# Autodesk Inventor assembly: Schwingforderer SF-TAG-N 250-20-105 R Al with loose ground(SRL-N250 AL)
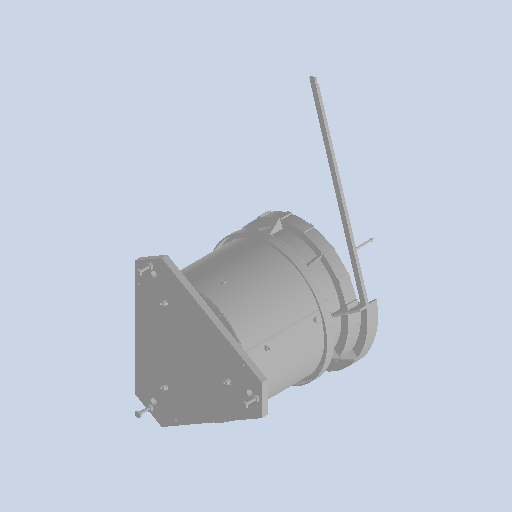
[picture p0: Inventor's stored thumbnail of the model, 512x512]
Saved by Autodesk Inventor 2025.2 (Build 292293000, 293)
## iProperties
Category: PARTsolutions
Company: RNA
Created: 2025-06-16
Part Number: Schwingforderer SF-TAG-N 250-20-105 R Al with loose ground(SRL-N250 AL)
Catalog Web Link: www.cadenas.de
Description: 250-Vibratory Bowl Feeder
Vendor: RNA
Document SubType Name: Assembly
Designer: psAdmin
Manufacturer: RNA
Mass: 8037.77 g
Surface Area: 14728.5 cm^2
Volume: 8037.77 cm^3
Density: 1 g/cm^3
PSOL_IDENT_0: {$CADENAS_DATA/23d-libs/rna/schwingfoerderer/bg_250.prj},262 {STYP=ASS},{VTYP=3D},{NB=Schwingfordere
PSOL_IDENT_1: r SF-TAG-N 250-20-105 R Al with loose ground(SRL-N250 AL)},{LINA=SF-TAG-N 250-20-105 R Al with loose
PSOL_IDENT_2: ground},{NN=250},{DATE=06.06.2017 07:12:53},{GEOMDATE=02.06.2017 06:00:57},{VERSION=},{LINEID=120},
PSOL_IDENT_3: {WBVAR=},{WBNUMERIC=}  {NB=Schwingforderer SF-TAG-N 250-20-105 R Al with loose ground(SRL-N250 AL)},
PSOL_IDENT_4: {LINA=SF-TAG-N 250-20-105 R Al with loose ground},{KT=DUMMY},{NAME=SF-TAG-N 250-20-105 R Al with loo
PSOL_IDENT_5: se ground},{INAME=SF2dTAG2dN202502d202d10520R20Al20with20loose20ground},{SHA256=rV/3CrsxDAyYqkcBF+Y8
PSOL_IDENT_6: nExrJVCtF3b6/2GE7EfEZ3w=},{CNSORDERNO=SF-TAG-N 250-20-105 R Al with loose ground},{HIDE=0},{A=Stufen
PSOL_IDENT_7: },{B=250},{C=Radial oben},{D=ALU},{E=Lose eingelegt},{F=20},{G=TAG-N250-20-105},{H=ohne},{I=SRL-N250
PSOL_IDENT_8: AL},{J=SRC-N250},{K=USJ250}
NB: Schwingforderer SF-TAG-N 250-20-105 R Al with loose ground(SRL-N250 AL)
NN: 250
NT: Vibratory Bowl Feeder
NBSYN: Schwingforderer $CNSORDERNO.($I.)
LINA: SF-TAG-N 250-20-105 R Al with loose ground
CATALOG: Rhein-Nadel-Automation
CNSORDERNO: SF-TAG-N 250-20-105 R Al with loose ground
A: Stufen
B: 250
C: Radial oben
D: ALU
E: Lose eingelegt
F: 20
G: TAG-N250-20-105
H: ohne
I: SRL-N250 AL
J: SRC-N250
K: USJ250
SUPPLIER: RNA
ARTICLENO: Schwingforderer SF-TAG-N 250-20-105 R Al with loose ground(SRL-N250 AL)
BOMINFO: SF-TAG-N 250-20-105 R Al with loose ground
CREATOR: CADENAS GmbH
Title: SF-TAG-N 250-20-105 R Al with loose ground
Author: Cadenas PARTsolutions
Comments: Vibratory Bowl Feeder
## Documents named in this file (40)
- D:\Useless_Box\CAD-Paspa\Useless Box\Kaufteile\SF-TAG-N 250-20-105 R Al\Schwingforderer SF-TAG-N 250-20-105 R Al with loose ground(SRL-N250 AL).iam
- D:\Useless_Box\CAD-Paspa\Useless Box\Kaufteile\SF-TAG-N 250-20-105 R Al\Schwingforderer SF-TAG-N 250-20-105 R Al with loose ground(SRL-N250 AL)_PART1.ipt
- D:\Useless_Box\CAD-Paspa\Useless Box\Kaufteile\SF-TAG-N 250-20-105 R Al\Schwingforderer SF-TAG-N 250-20-105 R Al with loose ground(SRL-N250 AL)_PART2.ipt
- D:\Useless_Box\CAD-Paspa\Useless Box\Kaufteile\SF-TAG-N 250-20-105 R Al\Schwingforderer SF-TAG-N 250-20-105 R Al with loose ground(SRL-N250 AL)_PART3.ipt
- D:\Useless_Box\CAD-Paspa\Useless Box\Kaufteile\SF-TAG-N 250-20-105 R Al\Schwingforderer SF-TAG-N 250-20-105 R Al with loose ground(SRL-N250 AL)_PART4.ipt
- D:\Useless_Box\CAD-Paspa\Useless Box\Kaufteile\SF-TAG-N 250-20-105 R Al\Schwingforderer SF-TAG-N 250-20-105 R Al with loose ground(SRL-N250 AL)_PART5.ipt
- D:\Useless_Box\CAD-Paspa\Useless Box\Kaufteile\SF-TAG-N 250-20-105 R Al\Schwingforderer SF-TAG-N 250-20-105 R Al with loose ground(SRL-N250 AL)_PART6.ipt
- D:\Useless_Box\CAD-Paspa\Useless Box\Kaufteile\SF-TAG-N 250-20-105 R Al\Schwingforderer SF-TAG-N 250-20-105 R Al with loose ground(SRL-N250 AL)_PART7.ipt
- D:\Useless_Box\CAD-Paspa\Useless Box\Kaufteile\SF-TAG-N 250-20-105 R Al\Schwingforderer SF-TAG-N 250-20-105 R Al with loose ground(SRL-N250 AL)_PART8.ipt
- D:\Useless_Box\CAD-Paspa\Useless Box\Kaufteile\SF-TAG-N 250-20-105 R Al\Schwingforderer SF-TAG-N 250-20-105 R Al with loose ground(SRL-N250 AL)_PART9.ipt
- D:\Useless_Box\CAD-Paspa\Useless Box\Kaufteile\SF-TAG-N 250-20-105 R Al\Schwingforderer SF-TAG-N 250-20-105 R Al with loose ground(SRL-N250 AL)_PART10.ipt
- D:\Useless_Box\CAD-Paspa\Useless Box\Kaufteile\SF-TAG-N 250-20-105 R Al\Schwingforderer SF-TAG-N 250-20-105 R Al with loose ground(SRL-N250 AL)_PART11.ipt
- D:\Useless_Box\CAD-Paspa\Useless Box\Kaufteile\SF-TAG-N 250-20-105 R Al\Schwingforderer SF-TAG-N 250-20-105 R Al with loose ground(SRL-N250 AL)_PART12.ipt
- D:\Useless_Box\CAD-Paspa\Useless Box\Kaufteile\SF-TAG-N 250-20-105 R Al\Schwingforderer SF-TAG-N 250-20-105 R Al with loose ground(SRL-N250 AL)_PART13.ipt
- D:\Useless_Box\CAD-Paspa\Useless Box\Kaufteile\SF-TAG-N 250-20-105 R Al\Schwingforderer SF-TAG-N 250-20-105 R Al with loose ground(SRL-N250 AL)_PART14.ipt
- D:\Useless_Box\CAD-Paspa\Useless Box\Kaufteile\SF-TAG-N 250-20-105 R Al\Schwingforderer SF-TAG-N 250-20-105 R Al with loose ground(SRL-N250 AL)_PART15.ipt
- D:\Useless_Box\CAD-Paspa\Useless Box\Kaufteile\SF-TAG-N 250-20-105 R Al\Schwingforderer SF-TAG-N 250-20-105 R Al with loose ground(SRL-N250 AL)_PART16.ipt
- D:\Useless_Box\CAD-Paspa\Useless Box\Kaufteile\SF-TAG-N 250-20-105 R Al\Schwingforderer SF-TAG-N 250-20-105 R Al with loose ground(SRL-N250 AL)_PART17.ipt
- D:\Useless_Box\CAD-Paspa\Useless Box\Kaufteile\SF-TAG-N 250-20-105 R Al\Schwingforderer SF-TAG-N 250-20-105 R Al with loose ground(SRL-N250 AL)_PART18.ipt
- D:\Useless_Box\CAD-Paspa\Useless Box\Kaufteile\SF-TAG-N 250-20-105 R Al\Schwingforderer SF-TAG-N 250-20-105 R Al with loose ground(SRL-N250 AL)_PART19.ipt
- D:\Useless_Box\CAD-Paspa\Useless Box\Kaufteile\SF-TAG-N 250-20-105 R Al\Schwingforderer SF-TAG-N 250-20-105 R Al with loose ground(SRL-N250 AL)_PART20.ipt
- D:\Useless_Box\CAD-Paspa\Useless Box\Kaufteile\SF-TAG-N 250-20-105 R Al\Schwingforderer SF-TAG-N 250-20-105 R Al with loose ground(SRL-N250 AL)_PART21.ipt
- D:\Useless_Box\CAD-Paspa\Useless Box\Kaufteile\SF-TAG-N 250-20-105 R Al\Schwingforderer SF-TAG-N 250-20-105 R Al with loose ground(SRL-N250 AL)_PART22.ipt
- D:\Useless_Box\CAD-Paspa\Useless Box\Kaufteile\SF-TAG-N 250-20-105 R Al\Schwingforderer SF-TAG-N 250-20-105 R Al with loose ground(SRL-N250 AL)_PART23.ipt
- D:\Useless_Box\CAD-Paspa\Useless Box\Kaufteile\SF-TAG-N 250-20-105 R Al\Schwingforderer SF-TAG-N 250-20-105 R Al with loose ground(SRL-N250 AL)_PART24.ipt
- D:\Useless_Box\CAD-Paspa\Useless Box\Kaufteile\SF-TAG-N 250-20-105 R Al\Schwingforderer SF-TAG-N 250-20-105 R Al with loose ground(SRL-N250 AL)_PART25.ipt
- D:\Useless_Box\CAD-Paspa\Useless Box\Kaufteile\SF-TAG-N 250-20-105 R Al\Schwingforderer SF-TAG-N 250-20-105 R Al with loose ground(SRL-N250 AL)_PART26.ipt
- D:\Useless_Box\CAD-Paspa\Useless Box\Kaufteile\SF-TAG-N 250-20-105 R Al\Schwingforderer SF-TAG-N 250-20-105 R Al with loose ground(SRL-N250 AL)_PART27.ipt
- D:\Useless_Box\CAD-Paspa\Useless Box\Kaufteile\SF-TAG-N 250-20-105 R Al\Schwingforderer SF-TAG-N 250-20-105 R Al with loose ground(SRL-N250 AL)_PART28.ipt
- D:\Useless_Box\CAD-Paspa\Useless Box\Kaufteile\SF-TAG-N 250-20-105 R Al\Schwingforderer SF-TAG-N 250-20-105 R Al with loose ground(SRL-N250 AL)_PART29.ipt
- D:\Useless_Box\CAD-Paspa\Useless Box\Kaufteile\SF-TAG-N 250-20-105 R Al\Schwingforderer SF-TAG-N 250-20-105 R Al with loose ground(SRL-N250 AL)_PART30.ipt
- D:\Useless_Box\CAD-Paspa\Useless Box\Kaufteile\SF-TAG-N 250-20-105 R Al\Schwingforderer SF-TAG-N 250-20-105 R Al with loose ground(SRL-N250 AL)_PART31.ipt
- D:\Useless_Box\CAD-Paspa\Useless Box\Kaufteile\SF-TAG-N 250-20-105 R Al\Schwingforderer SF-TAG-N 250-20-105 R Al with loose ground(SRL-N250 AL)_PART32.ipt
- D:\Useless_Box\CAD-Paspa\Useless Box\Kaufteile\SF-TAG-N 250-20-105 R Al\Schwingforderer SF-TAG-N 250-20-105 R Al with loose ground(SRL-N250 AL)_PART33.ipt
- D:\Useless_Box\CAD-Paspa\Useless Box\Kaufteile\SF-TAG-N 250-20-105 R Al\Schwingforderer SF-TAG-N 250-20-105 R Al with loose ground(SRL-N250 AL)_PART34.ipt
- D:\Useless_Box\CAD-Paspa\Useless Box\Kaufteile\SF-TAG-N 250-20-105 R Al\Schwingforderer SF-TAG-N 250-20-105 R Al with loose ground(SRL-N250 AL)_PART35.ipt
- D:\Useless_Box\CAD-Paspa\Useless Box\Kaufteile\SF-TAG-N 250-20-105 R Al\Schwingforderer SF-TAG-N 250-20-105 R Al with loose ground(SRL-N250 AL)_PART36.ipt
- D:\Useless_Box\CAD-Paspa\Useless Box\Kaufteile\SF-TAG-N 250-20-105 R Al\Schwingforderer SF-TAG-N 250-20-105 R Al with loose ground(SRL-N250 AL)_PART37.ipt
- D:\Useless_Box\CAD-Paspa\Useless Box\Kaufteile\SF-TAG-N 250-20-105 R Al\Schwingforderer SF-TAG-N 250-20-105 R Al with loose ground(SRL-N250 AL)_PART38.ipt
- D:\Useless_Box\CAD-Paspa\Useless Box\Kaufteile\IB06A229_ind_sensor\IB06A229.ipt
## Components (39 placed, 39 different names)
1. Schwingforderer SF-TAG-N 250-20-105 R Al with loose ground(SRL-N250 AL)_PART1:1
2. Schwingforderer SF-TAG-N 250-20-105 R Al with loose ground(SRL-N250 AL)_PART2:1
3. Schwingforderer SF-TAG-N 250-20-105 R Al with loose ground(SRL-N250 AL)_PART3:1
4. Schwingforderer SF-TAG-N 250-20-105 R Al with loose ground(SRL-N250 AL)_PART4:1
5. Schwingforderer SF-TAG-N 250-20-105 R Al with loose ground(SRL-N250 AL)_PART5:1
6. Schwingforderer SF-TAG-N 250-20-105 R Al with loose ground(SRL-N250 AL)_PART6:1
7. Schwingforderer SF-TAG-N 250-20-105 R Al with loose ground(SRL-N250 AL)_PART7:1
8. Schwingforderer SF-TAG-N 250-20-105 R Al with loose ground(SRL-N250 AL)_PART8:1
9. Schwingforderer SF-TAG-N 250-20-105 R Al with loose ground(SRL-N250 AL)_PART9:1
10. Schwingforderer SF-TAG-N 250-20-105 R Al with loose ground(SRL-N250 AL)_PART10:1
11. Schwingforderer SF-TAG-N 250-20-105 R Al with loose ground(SRL-N250 AL)_PART11:1
12. Schwingforderer SF-TAG-N 250-20-105 R Al with loose ground(SRL-N250 AL)_PART12:1 — Passend:1
13. Schwingforderer SF-TAG-N 250-20-105 R Al with loose ground(SRL-N250 AL)_PART13:1
14. Schwingforderer SF-TAG-N 250-20-105 R Al with loose ground(SRL-N250 AL)_PART14:1
15. Schwingforderer SF-TAG-N 250-20-105 R Al with loose ground(SRL-N250 AL)_PART15:1
16. Schwingforderer SF-TAG-N 250-20-105 R Al with loose ground(SRL-N250 AL)_PART16:1
17. Schwingforderer SF-TAG-N 250-20-105 R Al with loose ground(SRL-N250 AL)_PART17:1
18. Schwingforderer SF-TAG-N 250-20-105 R Al with loose ground(SRL-N250 AL)_PART18:1
19. Schwingforderer SF-TAG-N 250-20-105 R Al with loose ground(SRL-N250 AL)_PART19:1
20. Schwingforderer SF-TAG-N 250-20-105 R Al with loose ground(SRL-N250 AL)_PART20:1
21. Schwingforderer SF-TAG-N 250-20-105 R Al with loose ground(SRL-N250 AL)_PART21:1
22. Schwingforderer SF-TAG-N 250-20-105 R Al with loose ground(SRL-N250 AL)_PART22:1
23. Schwingforderer SF-TAG-N 250-20-105 R Al with loose ground(SRL-N250 AL)_PART23:1
24. Schwingforderer SF-TAG-N 250-20-105 R Al with loose ground(SRL-N250 AL)_PART24:1
25. Schwingforderer SF-TAG-N 250-20-105 R Al with loose ground(SRL-N250 AL)_PART25:1
26. Schwingforderer SF-TAG-N 250-20-105 R Al with loose ground(SRL-N250 AL)_PART26:1
27. Schwingforderer SF-TAG-N 250-20-105 R Al with loose ground(SRL-N250 AL)_PART27:1
28. Schwingforderer SF-TAG-N 250-20-105 R Al with loose ground(SRL-N250 AL)_PART28:1
29. Schwingforderer SF-TAG-N 250-20-105 R Al with loose ground(SRL-N250 AL)_PART29:1
30. Schwingforderer SF-TAG-N 250-20-105 R Al with loose ground(SRL-N250 AL)_PART30:1
31. Schwingforderer SF-TAG-N 250-20-105 R Al with loose ground(SRL-N250 AL)_PART31:1
32. Schwingforderer SF-TAG-N 250-20-105 R Al with loose ground(SRL-N250 AL)_PART32:1
33. Schwingforderer SF-TAG-N 250-20-105 R Al with loose ground(SRL-N250 AL)_PART33:1
34. Schwingforderer SF-TAG-N 250-20-105 R Al with loose ground(SRL-N250 AL)_PART34:1
35. Schwingforderer SF-TAG-N 250-20-105 R Al with loose ground(SRL-N250 AL)_PART35:1
36. Schwingforderer SF-TAG-N 250-20-105 R Al with loose ground(SRL-N250 AL)_PART36:1
37. Schwingforderer SF-TAG-N 250-20-105 R Al with loose ground(SRL-N250 AL)_PART37:1
38. Schwingforderer SF-TAG-N 250-20-105 R Al with loose ground(SRL-N250 AL)_PART38:1
39. IB06A229:1 — Passend:1
## Relationships (1: Mate 1)
- Passend:1 [Mate]: Schwingforderer SF-TAG-N 250-20-105 R Al with loose ground(SRL-N250 AL)_PART12:1 ↔ IB06A229:1
